# Autodesk Inventor assembly: Slew Bearing
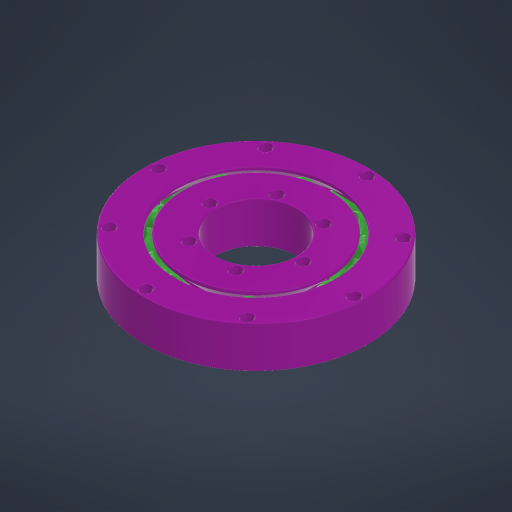
[picture p0: Inventor's stored thumbnail of the model, 512x512]
Saved by Autodesk Inventor 2023.1 (Build 271208000, 208)
## iProperties
Created: 2022-11-26
Part Number: Slew Bearing
Document SubType Name: Assembly
Designer: aubrey-work
Author: aubrey-work
## Documents named in this file (6)
- C:\GitHubRepos\PHYS-12-Website\content\portfolio\CAD Practice\Entries\1-Slew Bearing\Slew Bearing.iam
- C:\GitHubRepos\PHYS-12-Website\content\portfolio\CAD Practice\Entries\1-Slew Bearing\Roller.ipt
- C:\GitHubRepos\PHYS-12-Website\content\portfolio\CAD Practice\Entries\1-Slew Bearing\Track\Inner Track Bottom.ipt
- C:\GitHubRepos\PHYS-12-Website\content\portfolio\CAD Practice\Entries\1-Slew Bearing\Track\Inner Track Top.ipt
- C:\GitHubRepos\PHYS-12-Website\content\portfolio\CAD Practice\Entries\1-Slew Bearing\Track\Outer Track.ipt
- C:\GitHubRepos\PHYS-12-Website\content\portfolio\CAD Practice\Entries\1-Slew Bearing\SlewBearingParameters.xlsx
## Components (19 placed, 4 different names)
1. Inner Track Bottom:1 — Mate:1, Mate:2, Mate:5, Flush:1
2. Inner Track Top:1 — Mate:3, Mate:5
3. Outer Track:1 — Mate:4, Flush:1, Mate:6, Mate:7, Mate:8, Mate:9
4. Roller:1 — Mate:6, Mate:7
5. Roller:3
6. Roller:4
7. Roller:5
8. Roller:6
9. Roller:7
10. Roller:8
11. Roller:9
12. Roller:2 — Mate:8, Mate:9
13. Roller:12
14. Roller:13
15. Roller:14
16. Roller:15
17. Roller:16
18. Roller:17
19. Roller:18
## Component patterns: (8 elements, first: Roller:1), (8 elements, first: Roller:2)
## Relationships (10: Mate 9, Flush 1)
- Mate:1: Inner Track Bottom:1
- Mate:2: Inner Track Bottom:1
- Mate:3: Inner Track Top:1
- Mate:4: Outer Track:1
- Mate:5: Inner Track Bottom:1 ↔ Inner Track Top:1
- Flush:1: Inner Track Bottom:1 ↔ Outer Track:1
- Mate:6: Outer Track:1 ↔ Roller:1
- Mate:7: Outer Track:1 ↔ Roller:1
- Mate:8: Outer Track:1 ↔ Roller:2
- Mate:9: Outer Track:1 ↔ Roller:2
## Named parameters: gap = 0.1 mm, airgap = 0.4 mm, wallgap = 0.8 mm, roller_num = 16, roller_outerDiameter = 8 mm, roller_diameter = 8 mm, bolt_num = 8, bolt_diameter = 3 mm, outerBolt_num = 8, outerBolt_diameter = 3 mm, innerBolt_num = 6, innerBolt_diameter = 3 mm, elephantsFoot = 0.4 mm
